# Autodesk Inventor assembly: BallShooter
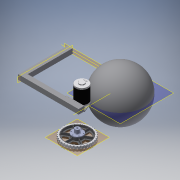
[picture p0: Inventor's stored thumbnail of the model, 180x180]
Saved by Autodesk Inventor 2016 SP1 (Build 200210100, 210)
## iProperties
Created: 2016-01-24
Part Number: BallShooter
Document SubType Name: Assembly
Designer: steele
Author: steele
## Documents named in this file (7)
- C:\snobotics\CAD-Development\robSteele\SnoBotics2016\2016-01-23-BallShooter\BallShooter.iam
- C:\snobotics\CAD-Development\robSteele\SnoBotics2016\2016-01-23-BallShooter\topOfFrame.ipt
- C:\snobotics\CAD-MfgResources\Andy-Mark\MotorMounts\AM 2488 CIM bracket.ipt
- C:\snobotics\CAD-MfgResources\Andy-Mark\Hubs\am-0320a_8mm_Key_Hub.ipt
- C:\snobotics\CAD-Development\robSteele\SnoBotics2016\DraftOfBoulder.ipt
- C:\snobotics\autodesk\2016\FRC KOP 2016\Motors\MOT_MiniCIMMotor_217-3371.ipt
- C:\snobotics\CAD-Development\robSteele\SnoBotics2016\2016-01-23-BallShooter\am-940a-6-HiGrip-.iam
## Components (6 placed, 6 different names)
1. topOfFrame:1 — Mate:4, Flush:1, Flush:2
2. AM 2488 CIM bracket:1 — Mate:4, Flush:1, Flush:2, Insert:4
3. MOT_MiniCIMMotor_217-3371:1 — Insert:4
4. am-0320a_8mm_Key_Hub:1 — Insert:5
5. am-940a-6-HiGrip-:1 [sub-assembly] — Insert:5
6. DraftOfBoulder:1 — Mate:2, Mate:3
## Relationships (7: Mate 3, Flush 2, Insert 2)
- Mate:2: DraftOfBoulder:1
- Mate:3: DraftOfBoulder:1
- Mate:4: topOfFrame:1 ↔ AM 2488 CIM bracket:1
- Flush:1: topOfFrame:1 ↔ AM 2488 CIM bracket:1
- Flush:2: topOfFrame:1 ↔ AM 2488 CIM bracket:1
- Insert:4: AM 2488 CIM bracket:1 ↔ MOT_MiniCIMMotor_217-3371:1
- Insert:5: am-0320a_8mm_Key_Hub:1 ↔ am-940a-6-HiGrip-:1
